# Autodesk Inventor assembly: SFU1605 Assem
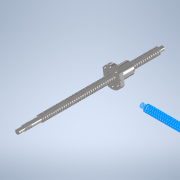
[picture p0: Inventor's stored thumbnail of the model, 180x180]
Saved by Autodesk Inventor 2021 (Build 250183000, 183)
## iProperties
Created: 2020-03-30
Part Number: SFU1605 Assem
Document SubType Name: Assembly
Designer: 79449
Sending System: SolidWorks 2020
Last Author: 79449
Last Saved: 2022-05-29
Author: 79449
## Documents named in this file (3)
- C:\Users\79449\Documents\CNC_DISENO_DE MAQUINAS\Piezas-Ensambles_Inventor\Segunda_presentación\SFU1605-1610\SFU1605 Assem.iam
- C:\Users\79449\Documents\CNC_DISENO_DE MAQUINAS\Piezas-Ensambles_Inventor\Segunda_presentación\SFU1605-1610\SFU1605-400.ipt
- C:\Users\79449\Documents\CNC_DISENO_DE MAQUINAS\Piezas-Ensambles_Inventor\Segunda_presentación\SFU1605-1610\SFU1605-1610.iam
## Components (2 placed, 2 different names)
1. SFU1605-400:1 — Cilíndrica:1
2. SFU1605-1610:2 [sub-assembly] — Cilíndrica:1
## Relationships (1: CylindricalJoint 1)
- Cilíndrica:1 [CylindricalJoint]: SFU1605-400:1 ↔ SFU1605-1610:2
